# Autodesk Inventor assembly: POM_T5_02
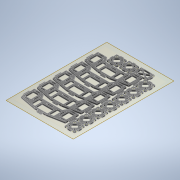
[picture p0: Inventor's stored thumbnail of the model, 180x180]
Saved by Autodesk Inventor 2022 (Build 260153000, 153)
## iProperties
Created: 2022-09-28
Part Number: POM_T5_02
Document SubType Name: Assembly
Designer: Masato
Author: Masato
## Documents named in this file (5)
- C:\Users\MasatoKubotera\Documents\Inventor\SUSTAINA-OP - CAM\Cam\POM_T5\OriginalMind_SR420\POM_T5_02.iam
- C:\Users\MasatoKubotera\Documents\Inventor\SUSTAINA-OP - CAM\Cam\DisposableBoard.ipt
- C:\Users\MasatoKubotera\Documents\Inventor\SUSTAINA-OP - CAM\UpperBody\Head\Head_neck_diagonal.ipt
- C:\Users\MasatoKubotera\Documents\Inventor\SUSTAINA-OP - CAM\UpperBody\Trunk\Trunk_chest_frame.iam
- C:\Users\MasatoKubotera\Documents\Inventor\SUSTAINA-OP - CAM\UpperBody\Arm\UpperArm_diagonal.ipt
## Components (16 placed, 4 different names)
1. DisposableBoard:1 — フラッシュ:1, フラッシュ:2, フラッシュ:3, フラッシュ:4, フラッシュ:9, フラッシュ:10, 角度:1
2. UpperArm_diagonal:8 — メイト:9, メイト:14, メイト:15, フラッシュ:14, 角度:1
3. UpperArm_diagonal:9 — メイト:10, フラッシュ:14, メイト:14, メイト:16, メイト:19
4. Head_neck_diagonal:1 — メイト:17, メイト:18, メイト:19
5. Trunk_chest_frame:1 [sub-assembly] — メイト:6, フラッシュ:9, フラッシュ:10, メイト:8, フラッシュ:11
6. Trunk_chest_frame:2 [sub-assembly]
7. Trunk_chest_frame:3 [sub-assembly]
8. Trunk_chest_frame:4 [sub-assembly]
9. Trunk_chest_frame:5 [sub-assembly] — メイト:15, メイト:16
10. UpperArm_diagonal:1 — メイト:7, メイト:8, フラッシュ:11
11. UpperArm_diagonal:2
12. UpperArm_diagonal:3
13. UpperArm_diagonal:4
14. UpperArm_diagonal:5
15. UpperArm_diagonal:6
16. UpperArm_diagonal:7 — メイト:18
## Component patterns: (5 elements, first: Trunk_chest_frame:1), (7 elements, first: UpperArm_diagonal:1)
## Relationships (20: Mate 11, Flush 8, Angle 1)
- フラッシュ:1 [Flush]: DisposableBoard:1
- フラッシュ:2 [Flush]: DisposableBoard:1
- フラッシュ:3 [Flush]: DisposableBoard:1
- フラッシュ:4 [Flush]: DisposableBoard:1
- メイト:6 [Mate]: Trunk_chest_frame:1
- フラッシュ:9 [Flush] (-2 mm): DisposableBoard:1 ↔ Trunk_chest_frame:1
- フラッシュ:10 [Flush] (-2 mm): DisposableBoard:1 ↔ Trunk_chest_frame:1
- メイト:7 [Mate]: UpperArm_diagonal:1
- メイト:8 [Mate] (2.1 mm): Trunk_chest_frame:1 ↔ UpperArm_diagonal:1
- フラッシュ:11 [Flush]: Trunk_chest_frame:1 ↔ UpperArm_diagonal:1
- メイト:9 [Mate]: UpperArm_diagonal:8
- メイト:10 [Mate]: UpperArm_diagonal:9
- フラッシュ:14 [Flush] (2.1 mm): UpperArm_diagonal:8 ↔ UpperArm_diagonal:9
- メイト:14 [Mate] (2.1 mm): UpperArm_diagonal:8 ↔ UpperArm_diagonal:9
- メイト:15 [Mate] (2.1 mm): UpperArm_diagonal:8 ↔ Trunk_chest_frame:5
- メイト:16 [Mate] (2.1 mm): UpperArm_diagonal:9 ↔ Trunk_chest_frame:5
- 角度:1 [Angle] (0 deg): DisposableBoard:1 ↔ UpperArm_diagonal:8
- メイト:17 [Mate]: Head_neck_diagonal:1
- メイト:18 [Mate] (2.1 mm): Head_neck_diagonal:1 ↔ UpperArm_diagonal:7
- メイト:19 [Mate] (2.1 mm): UpperArm_diagonal:9 ↔ Head_neck_diagonal:1
